# Autodesk Inventor assembly: スプリング
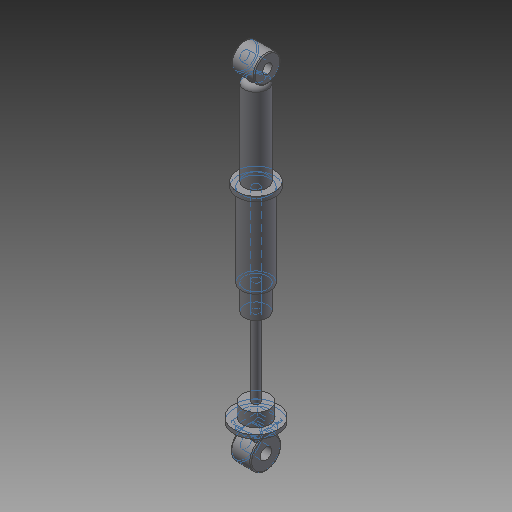
[picture p0: Inventor's stored thumbnail of the model, 512x512]
Saved by Autodesk Inventor 2018 (Build 220112000, 112)
## iProperties
Created: 2017-09-09
Part Number: スプリング
Material: 一般
Document SubType Name: Assembly
Designer: Kenta
Author: Kenta
## Documents named in this file (3)
- C:\Users\mura5\Documents\RBBR\cart\スプリング\スプリング.iam
- C:\Users\mura5\Documents\RBBR\cart\スプリング\スプリングその１.ipt
- C:\Users\mura5\Documents\RBBR\cart\スプリング\スプリングその２.ipt
## Components (2 placed, 2 different names)
1. スプリングその１:1 — メイト:1, メイト:2, 角度:1
2. スプリングその２:1 — メイト:1, メイト:2, 角度:1
## Relationships (3: Mate 2, Angle 1)
- メイト:1 [Mate]: スプリングその１:1 ↔ スプリングその２:1
- メイト:2 [Mate]: スプリングその１:1 ↔ スプリングその２:1
- 角度:1 [Angle] (0 deg): スプリングその１:1 ↔ スプリングその２:1
